# Autodesk Inventor assembly: 217-2778-001 Rev2_NCQ8A075-050M
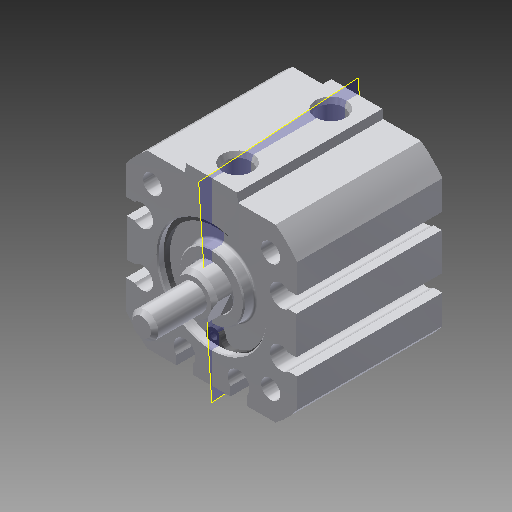
[picture p0: Inventor's stored thumbnail of the model, 512x512]
Saved by Autodesk Inventor 2017 (Build 210142000, 142)
## iProperties
Created: 2018-01-16
Part Number: 217-2778-001 Rev2_NCQ8A075-050M
Document SubType Name: Assembly
Designer: 600086
Mass: 19.858 g
Surface Area: 115.13 cm^2
Volume: 19.858 cm^3
Density: 1 g/cm^3
Author: 600086
Revision Number: ANY
## Documents named in this file (4)
- E:\GrabCAD\Power Hawks CAD\Resources\VEXpro Resources\Gearboxes\WCP shifting Gearbox\217-2778-001 Rev2_NCQ8A075-050M.iam
- E:\GrabCAD\Power Hawks CAD\Resources\VEXpro Resources\Gearboxes\WCP shifting Gearbox\217-2778-NCQ8A075-050M_NCQ8 Tube_075A.ipt
- E:\GrabCAD\Power Hawks CAD\Resources\VEXpro Resources\Gearboxes\WCP shifting Gearbox\217-2778-NCQ8A075-050M_NCQ8 Rod_075M.ipt
- E:\GrabCAD\Power Hawks CAD\Resources\VEXpro Resources\Gearboxes\WCP shifting Gearbox\217-2778-NCQ8A075-050M_Snap Ring_075.ipt
## Components (3 placed, 3 different names)
1. 217-2778-NCQ8A075-050M_NCQ8 Tube_075A_79 — Flush:1, Rigid:1, Rotational:1
2. 217-2778-NCQ8A075-050M_NCQ8 Rod_075M_80 — Rotational:1
3. 217-2778-NCQ8A075-050M_Snap Ring_075_81 — Rigid:1
## Relationships (3: Flush 1, WeldJoint 1, RevoluteJoint 1)
- Flush:1 (-15.875 mm): 217-2778-NCQ8A075-050M_NCQ8 Tube_075A_79
- Rigid:1 [WeldJoint]: 217-2778-NCQ8A075-050M_NCQ8 Tube_075A_79 ↔ 217-2778-NCQ8A075-050M_Snap Ring_075_81
- Rotational:1 [RevoluteJoint]: 217-2778-NCQ8A075-050M_NCQ8 Tube_075A_79 ↔ 217-2778-NCQ8A075-050M_NCQ8 Rod_075M_80
